# Autodesk Inventor assembly: Rocket
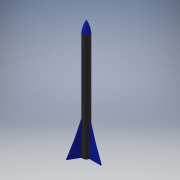
[picture p0: Inventor's stored thumbnail of the model, 180x180]
Saved by Autodesk Inventor 2018 (Build 220112000, 112)
## iProperties
Created: 2017-10-09
Part Number: Rocket
Document SubType Name: Assembly
Designer: Intel
Author: Intel
## Documents named in this file (6)
- C:\Users\Intel\git\GlencoeRocketz-2017\Inventor Files\Rocket.iam
- C:\Users\Intel\git\GlencoeRocketz-2017\Inventor Files\NoseCone.ipt
- C:\Users\Intel\git\GlencoeRocketz-2017\Inventor Files\Body.ipt
- C:\Users\Intel\git\GlencoeRocketz-2017\Inventor Files\Fin.ipt
- C:\Users\Intel\git\GlencoeRocketz-2017\Inventor Files\NoseCone_S2.ipt
- C:\Users\Intel\git\GlencoeRocketz-2017\Inventor Files\NoseCone_S3.ipt
## Components (7 placed, 5 different names)
1. NoseCone:1 — Mate:6, Mate:8
2. Body:1 — Mate:3, Flush:1, Tangent:1, Mate:4, Flush:2, Tangent:2, Mate:5, Flush:3, Tangent:3, Mate:10, Mate:11
3. Fin:1 — Mate:3, Flush:1, Tangent:1
4. Fin:2 — Mate:4, Flush:2, Tangent:2
5. Fin:3 — Mate:5, Flush:3, Tangent:3
6. NoseCone_S2:1 — Mate:6, Mate:7, Mate:8, Mate:9, Mate:11
7. NoseCone_S3:1 — Mate:7, Mate:9, Mate:10
## Relationships (15: Mate 9, Flush 3, Tangent 3)
- Mate:3: Body:1 ↔ Fin:1
- Flush:1: Body:1 ↔ Fin:1
- Tangent:1: Body:1 ↔ Fin:1
- Mate:4: Body:1 ↔ Fin:2
- Flush:2: Body:1 ↔ Fin:2
- Tangent:2: Body:1 ↔ Fin:2
- Mate:5: Body:1 ↔ Fin:3
- Flush:3: Body:1 ↔ Fin:3
- Tangent:3: Body:1 ↔ Fin:3
- Mate:6: NoseCone:1 ↔ NoseCone_S2:1
- Mate:7: NoseCone_S2:1 ↔ NoseCone_S3:1
- Mate:8: NoseCone:1 ↔ NoseCone_S2:1
- Mate:9: NoseCone_S2:1 ↔ NoseCone_S3:1
- Mate:10: Body:1 ↔ NoseCone_S3:1
- Mate:11: Body:1 ↔ NoseCone_S2:1
